# Autodesk Inventor assembly: GE-12088
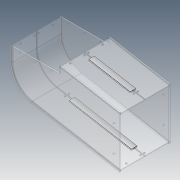
[picture p0: Inventor's stored thumbnail of the model, 180x180]
Saved by Autodesk Inventor 2012 (Build 160160000, 160)
## iProperties
Created: 2011-10-10
Part Number: GE-12088
Document SubType Name: Assembly
Designer: dfoster
Description: Chute 2 Assembly
Title: Chute 2 Assembly
Author: dfoster
## Documents named in this file (5)
- C:\Data Folder\FRC 2012 Field\Components\GE-12088.iam
- C:\Data Folder\FRC 2012 Field\Components\GE-12086.iam
- C:\Data Folder\FRC 2012 Field\Components\GE-12087.iam
- C:\Data Folder\FRC 2012 Field\Components\GE-12088-01.ipt
- C:\Data Folder\FRC 2012 Field\Components\GE-12088-02.ipt
## Components (4 placed, 4 different names)
1. GE-12086:1 [sub-assembly] — Mate:1, Flush:1, Flush:2, Mate:2
2. GE-12087:1 [sub-assembly] — Mate:1, Flush:1, Flush:2, Mate:3, Mate:4, Mate:5, Mate:6, Mate:7
3. GE-12088-01:1 — Mate:2, Mate:3, Mate:4
4. GE-12088-02:1 — Mate:5, Mate:6, Mate:7
## Relationships (9: Mate 7, Flush 2)
- Mate:1 (3.175 mm): GE-12086:1 ↔ GE-12087:1
- Flush:1: GE-12086:1 ↔ GE-12087:1
- Flush:2: GE-12086:1 ↔ GE-12087:1
- Mate:2: GE-12086:1 ↔ GE-12088-01:1
- Mate:3: GE-12087:1 ↔ GE-12088-01:1
- Mate:4 (57.15 mm): GE-12087:1 ↔ GE-12088-01:1
- Mate:5: GE-12087:1 ↔ GE-12088-02:1
- Mate:6: GE-12087:1 ↔ GE-12088-02:1
- Mate:7 (50.8 mm): GE-12087:1 ↔ GE-12088-02:1
